# Autodesk Inventor assembly: Lisbeth
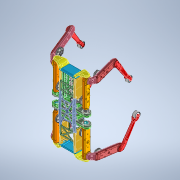
[picture p0: Inventor's stored thumbnail of the model, 180x180]
Saved by Autodesk Inventor 2022.2 (Build 262287000, 287)
## iProperties
Created: 2022-01-14
Part Number: Lisbeth
Document SubType Name: Assembly
Designer: Jochen
Author: Jochen
## Documents named in this file (5)
- D:\Projects\Lisbeth\CAD\Lisbeth.iam
- D:\Projects\Lisbeth\CAD\BodyStructure.iam
- D:\Projects\Lisbeth\CAD\Leg Long.iam
- D:\Projects\Lisbeth\CAD\Leg Short.iam
- D:\Projects\Lisbeth\CAD\Common\odrive\ODrive Pack.iam
## Components (6 placed, 4 different names)
1. BodyStructure:1 [sub-assembly] — Mate:20, Mate:21, Mate:22, Mate:23, Mate:24, Mate:25, Mate:26, Mate:27, Mate:29, Mate:30, Mate:31
2. ODrive Pack:1 [sub-assembly] — Mate:29, Mate:30, Mate:31
3. Leg Long:1 [sub-assembly] — Mate:22, Mate:23
4. Leg Long:2 [sub-assembly] — Mate:26, Mate:27
5. Leg Short:1 [sub-assembly] — Mate:20, Mate:21
6. Leg Short:2 [sub-assembly] — Mate:24, Mate:25
## Relationships (11: Mate 11)
- Mate:20: BodyStructure:1 ↔ Leg Short:1
- Mate:21: BodyStructure:1 ↔ Leg Short:1
- Mate:22: BodyStructure:1 ↔ Leg Long:1
- Mate:23: BodyStructure:1 ↔ Leg Long:1
- Mate:24: BodyStructure:1 ↔ Leg Short:2
- Mate:25: BodyStructure:1 ↔ Leg Short:2
- Mate:26: BodyStructure:1 ↔ Leg Long:2
- Mate:27: BodyStructure:1 ↔ Leg Long:2
- Mate:29: BodyStructure:1 ↔ ODrive Pack:1
- Mate:30 (1 mm): BodyStructure:1 ↔ ODrive Pack:1
- Mate:31 (2 mm): BodyStructure:1 ↔ ODrive Pack:1
